# Autodesk Inventor assembly: RadIntern
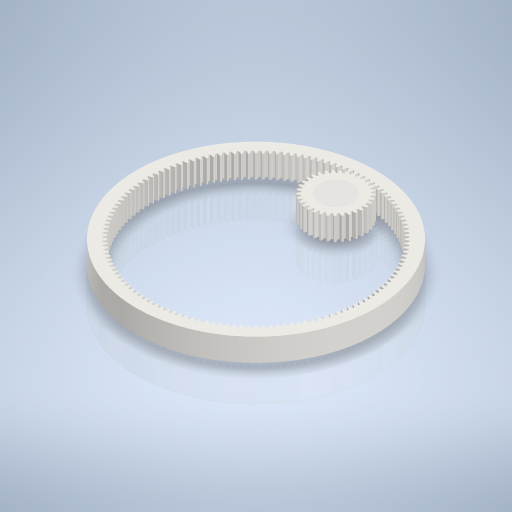
[picture p0: Inventor's stored thumbnail of the model, 512x512]
Saved by Autodesk Inventor 2024 (Build 280153000, 153)
## iProperties
Created: 2024-07-15
Part Number: RadIntern
Document SubType Name: Assembly
Designer: ffogue
Author: ffogue
## Documents named in this file (3)
- C:\Users\ffogue\OneDrive - MuM - OM\Dokumente\Inventor\Boxermotor\RadIntern.iam
- C:\Users\ffogue\OneDrive - MuM - OM\Dokumente\Inventor\Boxermotor\RadIntern\Konstruktions-Assistent\Stirnräder1.iam
- C:\Users\ffogue\OneDrive - MuM - OM\Dokumente\Inventor\Boxermotor\FüllungRad_10.ipt
## Components (2 placed, 2 different names)
1. Stirnräder:1 [sub-assembly] — Passend:1, Fluchtend:1
2. FüllungRad_10:1 — Passend:1, Fluchtend:1
## Relationships (2: Mate 1, Flush 1)
- Passend:1 [Mate]: Stirnräder:1 ↔ FüllungRad_10:1
- Fluchtend:1 [Flush]: Stirnräder:1 ↔ FüllungRad_10:1
